# Autodesk Inventor assembly: RoboticArm
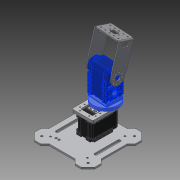
[picture p0: Inventor's stored thumbnail of the model, 180x180]
Saved by Autodesk Inventor 2018 (Build 220112000, 112)
## iProperties
Created: 2021-01-26
Part Number: RoboticArm
Material: Ogólny
Document SubType Name: Assembly
Designer: Marzena
Mass: 128.647 g
Surface Area: 583.737 cm^2
Volume: 128.647 cm^3
Density: 1 g/cm^3
Author: Marzena
## Documents named in this file (4)
- C:\Users\Marzena\Desktop\InventorArduinoC#\PhantomX Pincher Robot Arm\RoboticArm.iam
- C:\Users\Marzena\Desktop\InventorArduinoC#\PhantomX Pincher Robot Arm\Zespół1_Shrinkwrap_1.ipt
- C:\Users\Marzena\Desktop\InventorArduinoC#\PhantomX Pincher Robot Arm\Zespół2_Shrinkwrap_1.ipt
- C:\Users\Marzena\Desktop\InventorArduinoC#\PhantomX Pincher Robot Arm\f4Bracket.ipt
## Components (3 placed, 3 different names)
1. Zespół1_Shrinkwrap_1:1 — Wstaw:1, asd
2. Zespół2_Shrinkwrap_1:1 — Wstaw:1, asd, Obrotowe:1
3. f4Bracket:1 — Obrotowe:1
## Relationships (3: Insert 1, CylindricalJoint 1, RevoluteJoint 1)
- Wstaw:1 [Insert]: Zespół1_Shrinkwrap_1:1 ↔ Zespół2_Shrinkwrap_1:1
- asd [CylindricalJoint]: Zespół1_Shrinkwrap_1:1 ↔ Zespół2_Shrinkwrap_1:1
- Obrotowe:1 [RevoluteJoint]: Zespół2_Shrinkwrap_1:1 ↔ f4Bracket:1
